# Autodesk Inventor assembly: coveyer belt
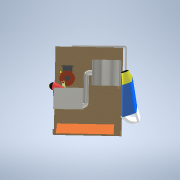
[picture p0: Inventor's stored thumbnail of the model, 180x180]
Saved by Autodesk Inventor 2021 (Build 250183000, 183)
## iProperties
Created: 2021-07-01
Part Number: coveyer belt
Document SubType Name: Assembly
Designer: HP
Author: HP
## Documents named in this file (16)
- D:\exploration\virtual\virtual\Final Assembly.iam
- D:\exploration\virtual\virtual\Base model.ipt
- D:\exploration\virtual\Wheel slider 1.2\base stand.ipt
- D:\exploration\virtual\Wheel slider 1.2\wheel 1.2.ipt
- D:\exploration\virtual\Wheel slider 1.2\T-shape 1.3.ipt
- D:\exploration\virtual\virtual\mould (1).ipt
- D:\exploration\virtual\virtual\Container 1.iam
- D:\exploration\virtual\virtual\air blower.ipt
- D:\exploration\virtual\virtual\vaccume.ipt
- D:\exploration\virtual\virtual\Slope.ipt
- D:\exploration\virtual\virtual\Dc motor.ipt
- D:\exploration\virtual\virtual\fan blade.ipt
- D:\exploration\virtual\virtual\cube bucket.ipt
- D:\exploration\virtual\virtual\cube lid.ipt
- D:\exploration\virtual\virtual\Servo motor.ipt
- D:\exploration\virtual\virtual\Pipe 1.4.ipt
## Components (16 placed, 15 different names)
1. Base model:1 — Rigid:1, Mate:5, Mate:6, Mate:7, Mate:8, Mate:15
2. base stand:1 — Rigid:1, MECH 1
3. wheel 1.2:1 — Mate:3, Mate:4, MECH 1
4. T-shape 1.3:1 — Mate:3, Mate:4, Rigid:2
5. mould (1):1 — Rigid:2
6. Container 1:1 [sub-assembly] — Mate:5, Mate:9, Rigid:3
7. air blower:1 — Mate:10
8. vaccume:1 — Mate:6
9. Slope:1 — Mate:7, Mate:8
10. Dc motor:1 — DC MOTOR, Mate:9
11. fan blade:1 — DC MOTOR
12. cube bucket:1 — Rigid:3, LID ROTATION, Mate:10, Mate:11, Mate:12
13. cube lid:1 — LID ROTATION, Mate:13, Mate:14
14. Servo motor:1 — Mate:11, Mate:12
15. mould (1):2 — Mate:13, Mate:14
16. Pipe 1.4:1 — Mate:15
## Relationships (19: Mate 13, WeldJoint 3, RevoluteJoint 3)
- Rigid:1 [WeldJoint]: Base model:1 ↔ base stand:1
- Mate:3: wheel 1.2:1 ↔ T-shape 1.3:1
- Mate:4: wheel 1.2:1 ↔ T-shape 1.3:1
- Rigid:2 [WeldJoint]: T-shape 1.3:1 ↔ mould (1):1
- Mate:5: Base model:1 ↔ Container 1:1
- Mate:6: Base model:1 ↔ vaccume:1
- Mate:7: Base model:1 ↔ Slope:1
- Mate:8: Base model:1 ↔ Slope:1
- MECH 1 [RevoluteJoint]: base stand:1 ↔ wheel 1.2:1
- DC MOTOR [RevoluteJoint]: Dc motor:1 ↔ fan blade:1
- Mate:9: Container 1:1 ↔ Dc motor:1
- Rigid:3 [WeldJoint]: Container 1:1 ↔ cube bucket:1
- LID ROTATION [RevoluteJoint]: cube bucket:1 ↔ cube lid:1
- Mate:10: air blower:1 ↔ cube bucket:1
- Mate:11: cube bucket:1 ↔ Servo motor:1
- Mate:12: cube bucket:1 ↔ Servo motor:1
- Mate:13: cube lid:1 ↔ mould (1):2
- Mate:14 (950 mm): cube lid:1 ↔ mould (1):2
- Mate:15: Base model:1 ↔ Pipe 1.4:1
